# Autodesk Inventor assembly: PancakeGeneratorAlt
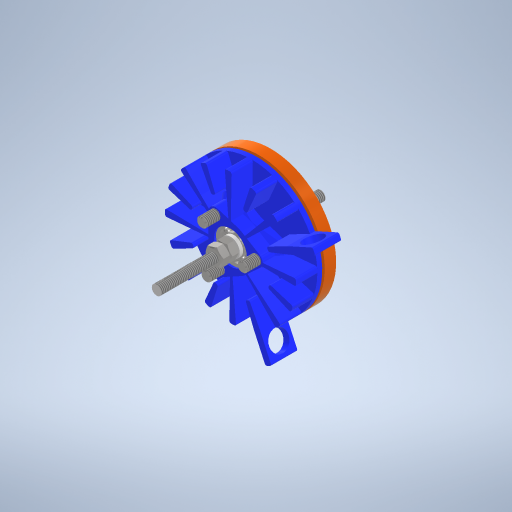
[picture p0: Inventor's stored thumbnail of the model, 512x512]
Saved by Autodesk Inventor 2024.3 (Build 283343000, 343)
## iProperties
Created: 2024-11-27
Part Number: PancakeGeneratorAlt
Document SubType Name: Assembly
Designer: Maximilian Hock
Author: Maximilian Hock
## Documents named in this file (8)
- Z:\Dokumente\LearningKit\LearningKitGenerator\PancakeGenerator.iam
- Z:\Dokumente\LearningKit\LearningKitGenerator\Axle.ipt
- Z:\Dokumente\LearningKit\LearningKitGenerator\PancakeRotor.ipt
- Z:\Dokumente\LearningKit\LearningKitGenerator\PancakeBearingAdapter.ipt
- Z:\Dokumente\LearningKit\LearningKitGenerator\PancakeStator.ipt
- Z:\Dokumente\Inventor\Content Center Files\R2024\de-DE\SKF - Single row ball bearings\SKF608.ipt
- Z:\Dokumente\Inventor\Content Center Files\R2024\de-DE\DIN EN ISO 4032\DIN EN ISO 4032 - M6.ipt
- Z:\Dokumente\Inventor\Content Center Files\R2024\de-DE\DIN EN ISO 4017\DIN EN ISO 4017 - M6 x 20.ipt
## Components (15 placed, 7 different names)
1. SKF- Kugellager, einreihig SKF608:3 — Starr:26, Starr:27, Drehbar:14
2. Axle:1 — Zylindrisch:9
3. PancakeRotor:1
4. DIN EN ISO 4032 M6:1
5. DIN EN ISO 4032 M6:2
6. DIN EN ISO 4032 M6:3
7. SKF- Kugellager, einreihig SKF608:4 — Starr:27
8. PancakeBearingAdapter:3 — Zylindrisch:9, Drehbar:14
9. PancakeStator:1 — Starr:26
10. DIN EN ISO 4017 M6 x 20:1
11. DIN EN ISO 4017 M6 x 20:2
12. DIN EN ISO 4017 M6 x 20:3
13. PancakeRotor:2
14. DIN EN ISO 4032 M6:4
15. DIN EN ISO 4032 M6:5
## Relationships (18: RevoluteJoint 6, CylindricalJoint 5, WeldJoint 4, PlanarJoint 3)
- [RevoluteJoint]: DIN EN ISO 4032 M6:2 ↔ DIN EN ISO 4032 M6:3
- Zylindrisch:9 [CylindricalJoint]: Axle:1 ↔ PancakeBearingAdapter:3
- [WeldJoint]: PancakeRotor:1 ↔ DIN EN ISO 4032 M6:1
- [RevoluteJoint]: DIN EN ISO 4032 M6:3 ↔ PancakeBearingAdapter:3
- [CylindricalJoint]: PancakeStator:1 ↔ DIN EN ISO 4017 M6 x 20:1
- [CylindricalJoint]: PancakeStator:1 ↔ DIN EN ISO 4017 M6 x 20:2
- [CylindricalJoint]: PancakeStator:1 ↔ DIN EN ISO 4017 M6 x 20:3
- [PlanarJoint]: PancakeStator:1 ↔ DIN EN ISO 4017 M6 x 20:3
- [PlanarJoint]: PancakeStator:1 ↔ DIN EN ISO 4017 M6 x 20:2
- [PlanarJoint]: PancakeStator:1 ↔ DIN EN ISO 4017 M6 x 20:1
- [WeldJoint]: DIN EN ISO 4032 M6:1 ↔ PancakeRotor:2
- [RevoluteJoint]: DIN EN ISO 4032 M6:4 ↔ DIN EN ISO 4032 M6:5
- [CylindricalJoint]: Axle:1 ↔ DIN EN ISO 4032 M6:4
- [RevoluteJoint]: PancakeRotor:2 ↔ DIN EN ISO 4032 M6:4
- Starr:26 [WeldJoint]: SKF- Kugellager, einreihig SKF608:3 ↔ PancakeStator:1
- Starr:27 [WeldJoint]: SKF- Kugellager, einreihig SKF608:3 ↔ SKF- Kugellager, einreihig SKF608:4
- Drehbar:14 [RevoluteJoint]: SKF- Kugellager, einreihig SKF608:3 ↔ PancakeBearingAdapter:3
- [RevoluteJoint]: DIN EN ISO 4032 M6:1 ↔ PancakeBearingAdapter:3
